# Autodesk Inventor assembly: prototype for arm
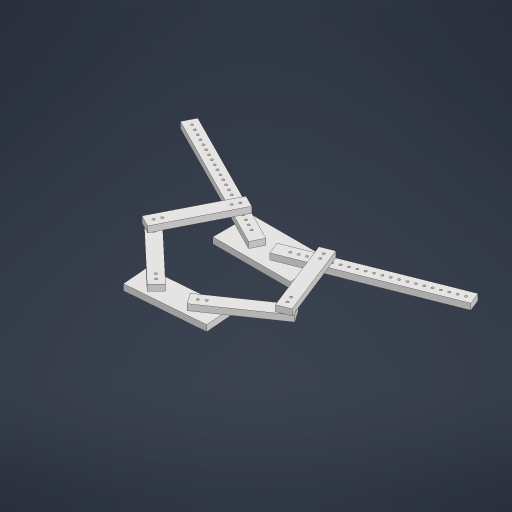
[picture p0: Inventor's stored thumbnail of the model, 512x512]
Saved by Autodesk Inventor 2023 (Build 270158000, 158)
## iProperties
Created: 2023-01-24
Part Number: prototype for arm
Document SubType Name: Assembly
Designer: Blank Slate
Author: Blank Slate
## Documents named in this file (5)
- C:\Users\Blank Slate\Documents\FRC 2023\prototype for arm.iam
- C:\Users\Blank Slate\Documents\FRC 2023\pincer2.0.ipt
- C:\Users\Blank Slate\Documents\FRC 2023\flat.ipt
- C:\Users\Blank Slate\Documents\FRC 2023\linkage.ipt
- C:\Users\Blank Slate\Documents\FRC 2023\track.ipt
## Components (8 placed, 4 different names)
1. pincer2.0:1 — Insert:2, Insert:6, Flush:2
2. pincer2.0:2 — Insert:1, Insert:5, Flush:3
3. flat:1 — Insert:1, Insert:2, Flush:1
4. linkage:1 — Mate:2, Insert:4
5. linkage:2 — Mate:2, Insert:6, Flush:2
6. linkage:3 — Mate:1, Insert:5, Flush:3
7. linkage:5 — Mate:1, Insert:3
8. track:1 — Flush:1, Insert:3, Insert:4
## Relationships (11: Insert 6, Flush 3, Mate 2)
- Insert:1: pincer2.0:2 ↔ flat:1
- Insert:2: pincer2.0:1 ↔ flat:1
- Mate:1: linkage:3 ↔ linkage:5
- Mate:2: linkage:1 ↔ linkage:2
- Flush:1: flat:1 ↔ track:1
- Insert:3: linkage:5 ↔ track:1
- Insert:4: linkage:1 ↔ track:1
- Insert:5: pincer2.0:2 ↔ linkage:3
- Insert:6: pincer2.0:1 ↔ linkage:2
- Flush:2: pincer2.0:1 ↔ linkage:2
- Flush:3: pincer2.0:2 ↔ linkage:3
